# Autodesk Inventor assembly: CNC_Cutting
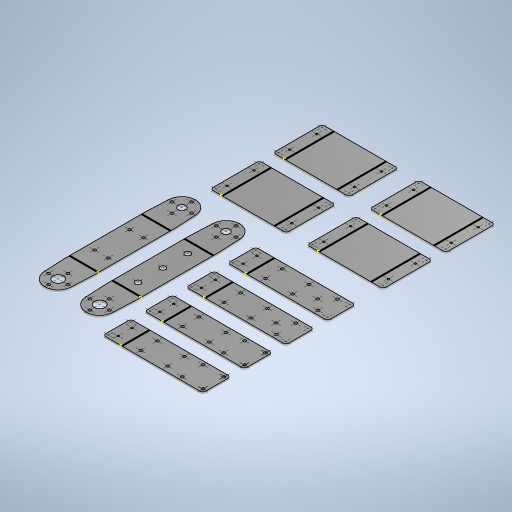
[picture p0: Inventor's stored thumbnail of the model, 512x512]
Saved by Autodesk Inventor 2023 (Build 270158000, 158)
## iProperties
Created: 2022-10-27
Part Number: CNC_Cutting
Document SubType Name: Assembly
Designer: chanh
Author: chanh
## Documents named in this file (6)
- C:\Users\chanh\OneDrive - 연세대학교 (Yonsei University)\로봇\Humanoid\Roboin Humanoid Project\Inventor\2-Axis Manipulator\Designs\Part\CAM\CNC_Cutting.iam
- C:\Users\chanh\OneDrive - 연세대학교 (Yonsei University)\로봇\Humanoid\Roboin Humanoid Project\Inventor\2-Axis Manipulator\Designs\Part\CAM\Part\CAM_servo_bracket_bottom.ipt
- C:\Users\chanh\OneDrive - 연세대학교 (Yonsei University)\로봇\Humanoid\Roboin Humanoid Project\Inventor\2-Axis Manipulator\Designs\Part\CAM\Part\CAM_servo_bracket_top.ipt
- C:\Users\chanh\OneDrive - 연세대학교 (Yonsei University)\로봇\Humanoid\Roboin Humanoid Project\Inventor\2-Axis Manipulator\Designs\Part\CAM\Part\CAM_ㄷ_frame_1.ipt
- C:\Users\chanh\OneDrive - 연세대학교 (Yonsei University)\로봇\Humanoid\Roboin Humanoid Project\Inventor\2-Axis Manipulator\Designs\Part\CAM\Part\CAM_ㄷ_frame_2.ipt
- C:\Users\chanh\OneDrive - 연세대학교 (Yonsei University)\로봇\Humanoid\Roboin Humanoid Project\Inventor\2-Axis Manipulator\Designs\Part\CAM\Part\CAM_ㄷ_frame_3.ipt
## Components (10 placed, 5 different names)
1. CAM_servo_bracket_bottom:1 — Flush:1, Flush:2, Mate:1, Flush:3, Mate:3, Flush:4, Flush:5, Mate:10
2. CAM_servo_bracket_bottom:2 — Mate:2, Flush:3, Mate:3, Mate:6
3. CAM_servo_bracket_top:2 — Mate:5, Flush:5, Mate:7, Mate:11, Mate:23, Flush:7
4. CAM_servo_bracket_top:1 — Mate:4, Flush:4, Mate:6, Mate:7
5. CAM_ㄷ_frame_1:1 — Mate:8, Mate:10, Mate:11, Mate:20, Mate:21
6. CAM_ㄷ_frame_3:1 — Mate:16, Flush:10, Mate:26
7. CAM_ㄷ_frame_3:2 — Mate:17, Mate:23, Flush:7, Mate:24, Flush:8, Flush:9, Mate:25
8. CAM_ㄷ_frame_3:3 — Mate:19, Mate:24, Flush:9, Flush:10, Mate:26
9. CAM_ㄷ_frame_3:4 — Mate:18, Flush:8, Mate:25
10. CAM_ㄷ_frame_2:1 — Mate:20, Mate:21, Mate:22
## Relationships (30: Mate 21, Flush 9)
- Flush:1: CAM_servo_bracket_bottom:1
- Flush:2: CAM_servo_bracket_bottom:1
- Mate:1: CAM_servo_bracket_bottom:1
- Mate:2: CAM_servo_bracket_bottom:2
- Flush:3: CAM_servo_bracket_bottom:1 ↔ CAM_servo_bracket_bottom:2
- Mate:3 (10 mm): CAM_servo_bracket_bottom:1 ↔ CAM_servo_bracket_bottom:2
- Mate:4: CAM_servo_bracket_top:1
- Mate:5: CAM_servo_bracket_top:2
- Flush:4: CAM_servo_bracket_bottom:1 ↔ CAM_servo_bracket_top:1
- Mate:6 (10 mm): CAM_servo_bracket_bottom:2 ↔ CAM_servo_bracket_top:1
- Flush:5: CAM_servo_bracket_bottom:1 ↔ CAM_servo_bracket_top:2
- Mate:7 (10 mm): CAM_servo_bracket_top:2 ↔ CAM_servo_bracket_top:1
- Mate:8: CAM_ㄷ_frame_1:1
- Mate:10 (10 mm): CAM_servo_bracket_bottom:1 ↔ CAM_ㄷ_frame_1:1
- Mate:11: CAM_servo_bracket_top:2 ↔ CAM_ㄷ_frame_1:1
- Mate:16: CAM_ㄷ_frame_3:1
- Mate:17: CAM_ㄷ_frame_3:2
- Mate:18: CAM_ㄷ_frame_3:4
- Mate:19: CAM_ㄷ_frame_3:3
- Mate:20 (10 mm): CAM_ㄷ_frame_1:1 ↔ CAM_ㄷ_frame_2:1
- Mate:21: CAM_ㄷ_frame_1:1 ↔ CAM_ㄷ_frame_2:1
- Mate:22: CAM_ㄷ_frame_2:1
- Mate:23 (20 mm): CAM_servo_bracket_top:2 ↔ CAM_ㄷ_frame_3:2
- Flush:7: CAM_servo_bracket_top:2 ↔ CAM_ㄷ_frame_3:2
- Mate:24 (10 mm): CAM_ㄷ_frame_3:2 ↔ CAM_ㄷ_frame_3:3
- Flush:8: CAM_ㄷ_frame_3:2 ↔ CAM_ㄷ_frame_3:4
- Flush:9: CAM_ㄷ_frame_3:2 ↔ CAM_ㄷ_frame_3:3
- Flush:10: CAM_ㄷ_frame_3:1 ↔ CAM_ㄷ_frame_3:3
- Mate:25 (15 mm): CAM_ㄷ_frame_3:2 ↔ CAM_ㄷ_frame_3:4
- Mate:26 (15 mm): CAM_ㄷ_frame_3:1 ↔ CAM_ㄷ_frame_3:3
